# Autodesk Inventor assembly: EL2-C-100
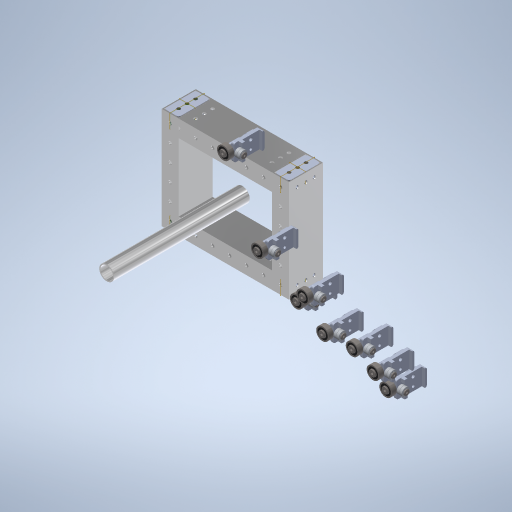
[picture p0: Inventor's stored thumbnail of the model, 512x512]
Saved by Autodesk Inventor 2023.4 (Build 274418000, 418)
## iProperties
Created: 2025-01-11
Part Number: EL2-C-100
Document SubType Name: Assembly
Designer: brand
Author: brand
## Documents named in this file (6)
- C:\Users\mavericks\Documents\Robotics\GitHub\2025-ReefScape---CAD\Elevator\EL2\EL2-C-100.iam
- C:\Users\mavericks\Documents\Robotics\GitHub\2025-ReefScape---CAD\Elevator\EL2\EL2-C-001.ipt
- C:\Users\mavericks\Documents\Robotics\GitHub\2025-ReefScape---CAD\Elevator\EL2\EL2-005.ipt
- C:\Users\mavericks\Documents\Robotics\GitHub\2025-ReefScape---CAD\Elevator\EL2\EL2-C-004.ipt
- C:\Users\mavericks\Documents\Robotics\GitHub\2025-ReefScape---CAD\Elevator\EL2\EL2-C-005.ipt
- C:\Users\mavericks\Documents\Robotics\GitHub\2025-ReefScape---CAD\COMMON PARTS\WCP Elevator parts\WCP-0323\WCP-0323.iam
## Components (17 placed, 5 different names)
1. EL2-C-001:1 — Flush:4, Flush:5, Flush:8, Mate:9, Mate:10, Flush:9, Flush:11
2. EL2-C-005:2 — Insert:1, Angle:1, Insert:2, Angle:2, Flush:4, Mate:10
3. EL2-C-005:1 — Insert:8, Angle:3, Insert:10, Angle:4, Flush:5, Mate:9, Mate:11
4. EL2-C-001:4 — Flush:10, Flush:11, Mate:11
5. EL2-005:1 — Insert:2, Angle:2, Flush:9
6. EL2-005:2 — Insert:8, Angle:3, Flush:8
7. EL2-005:3 — Insert:10, Angle:4, Flush:10
8. EL2-005:4 — Insert:1, Angle:1
9. EL2-C-004:1
10. WCP-0323:1 [sub-assembly]
11. WCP-0323:2 [sub-assembly]
12. WCP-0323:3 [sub-assembly]
13. WCP-0323:4 [sub-assembly]
14. WCP-0323:5 [sub-assembly]
15. WCP-0323:6 [sub-assembly]
16. WCP-0323:7 [sub-assembly]
17. WCP-0323:8 [sub-assembly]
## Relationships (17: Flush 6, Insert 4, Angle 4, Mate 3)
- Insert:1: EL2-C-005:2 ↔ EL2-005:4
- Angle:1 (0 deg): EL2-C-005:2 ↔ EL2-005:4
- Insert:2: EL2-C-005:2 ↔ EL2-005:1
- Angle:2 (0 deg): EL2-C-005:2 ↔ EL2-005:1
- Insert:8: EL2-C-005:1 ↔ EL2-005:2
- Angle:3 (0 deg): EL2-C-005:1 ↔ EL2-005:2
- Insert:10: EL2-C-005:1 ↔ EL2-005:3
- Angle:4 (0 deg): EL2-C-005:1 ↔ EL2-005:3
- Flush:4: EL2-C-001:1 ↔ EL2-C-005:2
- Flush:5: EL2-C-001:1 ↔ EL2-C-005:1
- Flush:8: EL2-C-001:1 ↔ EL2-005:2
- Mate:9: EL2-C-001:1 ↔ EL2-C-005:1
- Mate:10: EL2-C-001:1 ↔ EL2-C-005:2
- Flush:9: EL2-C-001:1 ↔ EL2-005:1
- Flush:10: EL2-C-001:4 ↔ EL2-005:3
- Flush:11: EL2-C-001:1 ↔ EL2-C-001:4
- Mate:11: EL2-C-005:1 ↔ EL2-C-001:4
